# Autodesk Inventor assembly: ASSY_REV,ENG_DESIGN2
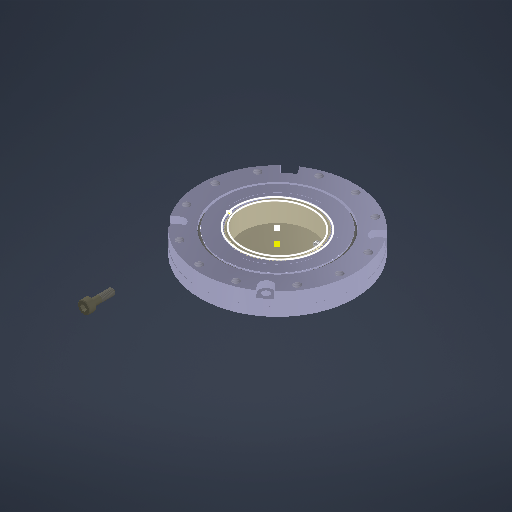
[picture p0: Inventor's stored thumbnail of the model, 512x512]
Saved by Autodesk Inventor 2026.2 (Build 302298010, 298A)
## iProperties
Created: 2026-02-10
Part Number: ASSY_REV,ENG_DESIGN2
Document SubType Name: Assembly
Designer: 4aida
Author: 4aida
## Documents named in this file (12)
- C:\Users\4aida\OneDrive\Documents\GitHub\Design_II_Group6\REV_ENG\ASSY_REV,ENG_DESIGN2.iam
- C:\Users\4aida\OneDrive\Documents\GitHub\Design_II_Group6\REV_ENG\ROLLER_CR_BEARING,REV-ENG.ipt
- C:\Users\4aida\OneDrive\Documents\GitHub\Design_II_Group6\REV_ENG\SPACER_ROLLER_CR_BEARING,REV-ENG.ipt
- C:\Users\4aida\OneDrive\Documents\GitHub\Design_II_Group6\REV_ENG\MIR_SPACER_ROLLER_CR_BEARING,REV-ENG.ipt
- C:\Users\4aida\OneDrive\Documents\GitHub\Design_II_Group6\REV_ENG\CR_ROLLER_BOUNDRY,REV-ENG.ipt
- C:\Users\4aida\OneDrive\Documents\GitHub\Design_II_Group6\REV_ENG\O_RING.ipt
- C:\Users\4aida\OneDrive\Documents\GitHub\Design_II_Group6\REV_ENG\CR_OUTSIDE,BOTTOM,REV-ENG.ipt
- C:\Users\4aida\OneDrive\Documents\GitHub\Design_II_Group6\REV_ENG\CR_OUTSIDE,TOP,REV-ENG.ipt
- C:\Users\4aida\OneDrive\Documents\GitHub\Design_II_Group6\REV_ENG\Fasteners\M3\SCREW,SOCKET-HD,P,12_9,M03X0_5X10MM.ipt
- C:\Users\4aida\OneDrive\Documents\GitHub\Design_II_Group6\REV_ENG\2.5mm_BALL_BEARINGS.ipt
- C:\Users\4aida\OneDrive\Documents\GitHub\Design_II_Group6\REV_ENG\Flex_SPLINE,REV-ENG.iam
- C:\Users\4aida\OneDrive\Documents\GitHub\Design_II_Group6\REV_ENG\DERIVEN_CR_INSIDE,REV-ENG.ipt
## Components (56 placed, 11 different names)
1. CR_ROLLER_BOUNDRY,REV-ENG:1 — Mate:23, Mate:24
2. O_RING:1 — Mate:16, Tangent:7
3. CR_OUTSIDE,BOTTOM,REV-ENG:1 — Mate:9, Mate:10, Mate:13, Flush:4
4. CR_OUTSIDE,TOP,REV-ENG:1 — Mate:9, Mate:10, Mate:12, Flush:6, Mate:17
5. SCREW,SOCKET-HD,P,12_9,M03X0_5X10MM:1
6. 2.5mm_BALL_BEARINGS:1 — Tangent:5, Tangent:6, Mate:14
7. Flex_SPLINE,REV-ENG:1 [sub-assembly] — Tangent:5, Tangent:6, Mate:14, Flush:5, Mate:15
8. DERIVEN_CR_INSIDE,REV-ENG:1 — Flush:5, Mate:15, Mate:16, Tangent:7, Flush:6, Mate:17, Mate:18, Mate:21, Tangent:8, Tangent:9
9. MIR_SPACER_ROLLER_CR_BEARING,REV-ENG:13 — Mate:21, Mate:22
10. ROLLER_CR_BEARING,REV-ENG:27 — Mate:20, Mate:22, Tangent:8
11. SPACER_ROLLER_CR_BEARING,REV-ENG:13 — Mate:18, Mate:19, Flush:7, Mate:20
12. ROLLER_CR_BEARING,REV-ENG:26 — Mate:19, Tangent:9
13. MIR_SPACER_ROLLER_CR_BEARING,REV-ENG:14
14. ROLLER_CR_BEARING,REV-ENG:28
15. SPACER_ROLLER_CR_BEARING,REV-ENG:14
16. ROLLER_CR_BEARING,REV-ENG:29
17. MIR_SPACER_ROLLER_CR_BEARING,REV-ENG:15
18. ROLLER_CR_BEARING,REV-ENG:30
19. SPACER_ROLLER_CR_BEARING,REV-ENG:15
20. ROLLER_CR_BEARING,REV-ENG:31
21. MIR_SPACER_ROLLER_CR_BEARING,REV-ENG:16
22. ROLLER_CR_BEARING,REV-ENG:32
23. SPACER_ROLLER_CR_BEARING,REV-ENG:16
24. ROLLER_CR_BEARING,REV-ENG:33
25. MIR_SPACER_ROLLER_CR_BEARING,REV-ENG:17
26. ROLLER_CR_BEARING,REV-ENG:34
27. SPACER_ROLLER_CR_BEARING,REV-ENG:17
28. ROLLER_CR_BEARING,REV-ENG:35
29. MIR_SPACER_ROLLER_CR_BEARING,REV-ENG:18
30. ROLLER_CR_BEARING,REV-ENG:36
31. SPACER_ROLLER_CR_BEARING,REV-ENG:18
32. ROLLER_CR_BEARING,REV-ENG:37
33. MIR_SPACER_ROLLER_CR_BEARING,REV-ENG:19
34. ROLLER_CR_BEARING,REV-ENG:38
35. SPACER_ROLLER_CR_BEARING,REV-ENG:19
36. ROLLER_CR_BEARING,REV-ENG:39
37. MIR_SPACER_ROLLER_CR_BEARING,REV-ENG:20
38. ROLLER_CR_BEARING,REV-ENG:40
39. SPACER_ROLLER_CR_BEARING,REV-ENG:20
40. ROLLER_CR_BEARING,REV-ENG:41
41. MIR_SPACER_ROLLER_CR_BEARING,REV-ENG:21
42. ROLLER_CR_BEARING,REV-ENG:42
43. SPACER_ROLLER_CR_BEARING,REV-ENG:21
44. ROLLER_CR_BEARING,REV-ENG:43
45. MIR_SPACER_ROLLER_CR_BEARING,REV-ENG:22
46. ROLLER_CR_BEARING,REV-ENG:44
47. SPACER_ROLLER_CR_BEARING,REV-ENG:22
48. ROLLER_CR_BEARING,REV-ENG:45
49. MIR_SPACER_ROLLER_CR_BEARING,REV-ENG:23
50. ROLLER_CR_BEARING,REV-ENG:46
51. SPACER_ROLLER_CR_BEARING,REV-ENG:23
52. ROLLER_CR_BEARING,REV-ENG:47
53. MIR_SPACER_ROLLER_CR_BEARING,REV-ENG:24
54. ROLLER_CR_BEARING,REV-ENG:48
55. SPACER_ROLLER_CR_BEARING,REV-ENG:24
56. ROLLER_CR_BEARING,REV-ENG:49
## Component patterns: (12 elements, first: MIR_SPACER_ROLLER_CR_BEARING,REV-ENG:13 + ROLLER_CR_BEARING,REV-ENG:27 + SPACER_ROLLER_CR_BEARING,REV-ENG:13 + ROLLER_CR_BEARING,REV-ENG:26)
## Relationships (24: Mate 15, Tangent 5, Flush 4)
- Mate:9: CR_OUTSIDE,BOTTOM,REV-ENG:1 ↔ CR_OUTSIDE,TOP,REV-ENG:1
- Mate:10: CR_OUTSIDE,BOTTOM,REV-ENG:1 ↔ CR_OUTSIDE,TOP,REV-ENG:1
- Tangent:5: 2.5mm_BALL_BEARINGS:1 ↔ Flex_SPLINE,REV-ENG:1
- Tangent:6: 2.5mm_BALL_BEARINGS:1 ↔ Flex_SPLINE,REV-ENG:1
- Mate:12: CR_OUTSIDE,TOP,REV-ENG:1
- Mate:13: CR_OUTSIDE,BOTTOM,REV-ENG:1
- Flush:4: CR_OUTSIDE,BOTTOM,REV-ENG:1
- Mate:14: 2.5mm_BALL_BEARINGS:1 ↔ Flex_SPLINE,REV-ENG:1
- Flush:5: Flex_SPLINE,REV-ENG:1 ↔ DERIVEN_CR_INSIDE,REV-ENG:1
- Mate:15: Flex_SPLINE,REV-ENG:1 ↔ DERIVEN_CR_INSIDE,REV-ENG:1
- Mate:16: O_RING:1 ↔ DERIVEN_CR_INSIDE,REV-ENG:1
- Tangent:7: O_RING:1 ↔ DERIVEN_CR_INSIDE,REV-ENG:1
- Flush:6: CR_OUTSIDE,TOP,REV-ENG:1 ↔ DERIVEN_CR_INSIDE,REV-ENG:1
- Mate:17: CR_OUTSIDE,TOP,REV-ENG:1 ↔ DERIVEN_CR_INSIDE,REV-ENG:1
- Mate:18: DERIVEN_CR_INSIDE,REV-ENG:1 ↔ SPACER_ROLLER_CR_BEARING,REV-ENG:13
- Mate:19: SPACER_ROLLER_CR_BEARING,REV-ENG:13 ↔ ROLLER_CR_BEARING,REV-ENG:26
- Flush:7: SPACER_ROLLER_CR_BEARING,REV-ENG:13
- Mate:20: ROLLER_CR_BEARING,REV-ENG:27 ↔ SPACER_ROLLER_CR_BEARING,REV-ENG:13
- Mate:21: DERIVEN_CR_INSIDE,REV-ENG:1 ↔ MIR_SPACER_ROLLER_CR_BEARING,REV-ENG:13
- Mate:22: MIR_SPACER_ROLLER_CR_BEARING,REV-ENG:13 ↔ ROLLER_CR_BEARING,REV-ENG:27
- Tangent:8 (0.125 mm): DERIVEN_CR_INSIDE,REV-ENG:1 ↔ ROLLER_CR_BEARING,REV-ENG:27
- Tangent:9 (0.125 mm): DERIVEN_CR_INSIDE,REV-ENG:1 ↔ ROLLER_CR_BEARING,REV-ENG:26
- Mate:23: CR_ROLLER_BOUNDRY,REV-ENG:1
- Mate:24: CR_ROLLER_BOUNDRY,REV-ENG:1
